# Autodesk Inventor assembly: KPA4CUNPL
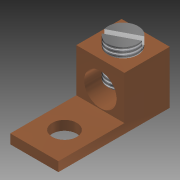
[picture p0: Inventor's stored thumbnail of the model, 180x180]
Saved by Autodesk Inventor 2014 (Build 180170000, 170)
## iProperties
Shininess: 64.0
Angle Display Precision: 2
Document Length Units: 11272
Document Angle Units: 11279
Document Time Units: 11290
Document Mass Units: 11286
Document Length Units Precision: 3
Document Angle Units Precision: 2
Category: Electrical
Company: Autodesk Inc.
Created: 2013-12-19
Part Number: KPA4CUNPL
Catalog Web Link: http://ecat.burndy.com/Comergent/en/US/adirect/fci?cmd=catProductDetail&showAddButton=true&productID=KPA4CUNPL&_bcs_=-1%08%23%23%08%23%23%08http%3A%2F%2Fecat.burndy.com%3A80%2FComergent%2Fen%2FUS%2Fadirect%2Ffci%3Fcmd%3DcatLanding%08%23%23%08true%08%07100%08kpa*%08Search%3Dkpa*%08%23%23%08%23%23%08false%08
Description: Terminal lug, 6-14ga solderless lug, mechanical
Vendor: FCI Burndy
Document SubType Name: Assembly
Designer: Autodesk Inc.
Density: 0.0
Volumn: 0.0
Area: 0.0
PropertySet Name: Model Information
Control State: 0
Master: False
Checked Out: False
Author: Autodesk Inc.
## Documents named in this file (3)
- D:\Data Folder\FIRST 2014\KOP Parts\Electrical\ELEC_Terminal Lug _KPA4CUNPL.iam
- D:\Data Folder\FIRST 2014\KOP Parts\Electrical\Parts\Terminal Battery.ipt
- D:\Data Folder\FIRST 2014\KOP Parts\Electrical\Parts\Terminal Screw.ipt
## Components (2 placed, 2 different names)
1. Terminal Battery:1 — Mate:1, Flush:1
2. Terminal Screw:1 — Mate:1, Flush:1
## Relationships (2: Mate 1, Flush 1)
- Mate:1: Terminal Battery:1 ↔ Terminal Screw:1
- Flush:1 (-2.54 mm): Terminal Battery:1 ↔ Terminal Screw:1
